# Autodesk Inventor assembly: ASY 940 linkage
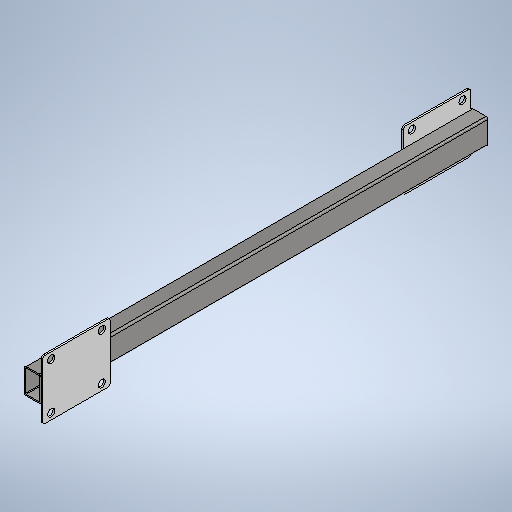
[picture p0: Inventor's stored thumbnail of the model, 512x512]
Saved by Autodesk Inventor 2025 (Build 290162010, 162A)
## iProperties
Created: 2024-09-11
Part Number: ASY 940 linkage
Document SubType Name: Assembly
Designer: admin
Author: admin
## Documents named in this file (3)
- C:\Users\admin\YandexDisk-badmisterfox\домашниий пк\Inventor\Manturovo\Manturovo_Se-clar\ASY 940 linkage.iam
- C:\Users\admin\YandexDisk-badmisterfox\домашниий пк\Inventor\Manturovo\Manturovo_Se-clar\ASY MSC 900.8 base frame transverse.ipt
- C:\Users\admin\YandexDisk-badmisterfox\домашниий пк\Inventor\Manturovo\Manturovo_Se-clar\ISO 657_14 - 60x40x3 - 1000.ipt
## Components (3 placed, 2 different names)
1. ASY MSC 900.8 base frame transverse:1
2. ASY MSC 900.8 base frame transverse:2
3. ISO 657_14 - 60x40x3 - 1000:1
## Relationships (2: WeldJoint 2)
- [WeldJoint]: ASY MSC 900.8 base frame transverse:2 ↔ ISO 657_14 - 60x40x3 - 1000:1
- [WeldJoint]: ASY MSC 900.8 base frame transverse:1 ↔ ISO 657_14 - 60x40x3 - 1000:1
